# Autodesk Inventor assembly: WormGearDriveForPot
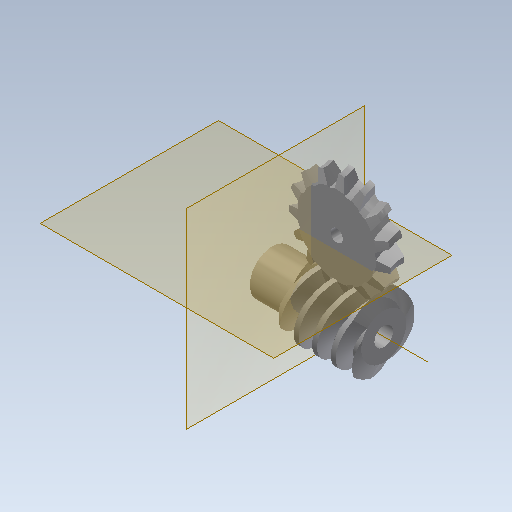
[picture p0: Inventor's stored thumbnail of the model, 512x512]
Saved by Autodesk Inventor 2020.2 (Build 242310000, 310)
## iProperties
Created: 2018-02-27
Part Number: WormGearDriveForPot
Document SubType Name: Assembly
Designer: steele
Author: steele
## Documents named in this file (4)
- C:\git\CAD-Development\robSteele\liftSpool\WormGearDriveForPot.iam
- C:\git\CAD-Development\robSteele\2018-FRC\Arm\blockToSupportShaftAndPot.ipt
- C:\git\CAD-Development\robSteele\2018-FRC\Arm\ShaftToConnectPotToMotor.ipt
- C:\git\CAD-Development\robSteele\liftSpool\PotHolderAssemblyWithWormGearDrive\Design Accelerator\Worm Gears1.iam
## Components (3 placed, 3 different names)
1. blockToSupportShaftAndPot:1 — Insert:3
2. ShaftToConnectPotToMotor:1 — Insert:3
3. Worm Gears:1 [sub-assembly]
## Relationships (1: Insert 1)
- Insert:3: blockToSupportShaftAndPot:1 ↔ ShaftToConnectPotToMotor:1
